# Autodesk Inventor assembly: 40-J4
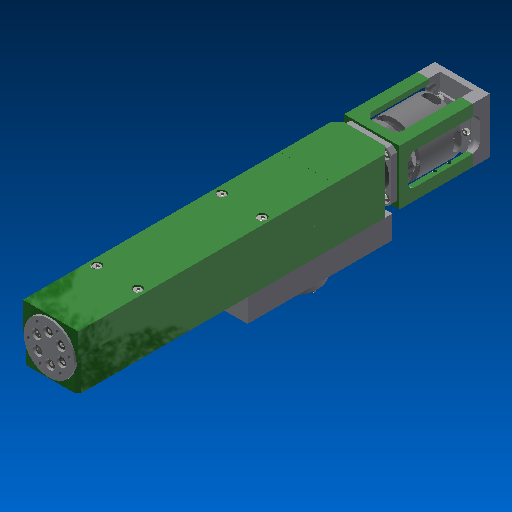
[picture p0: Inventor's stored thumbnail of the model, 512x512]
Saved by Autodesk Inventor 2018 (Build 220112000, 112)
## iProperties
Created: 2020-06-07
Part Number: 40-J4
Document SubType Name: Assembly
Designer: Bunny320
Author: Bunny320
## Documents named in this file (15)
- C:\Users\Bunny320\Desktop\sechs\4-CAD\40-J4.iam
- C:\Users\Bunny320\Desktop\sechs\4-CAD\motor unit 2820.iam
- C:\Users\Bunny320\Desktop\sechs\4-CAD\401-flange.ipt
- C:\Users\Bunny320\Desktop\sechs\4-CAD\402-gearbox-housing.ipt
- C:\Users\Bunny320\Desktop\sechs\4-CAD\403-coupler dummy.ipt
- C:\Users\Bunny320\Desktop\sechs\4-CAD\404-shaft.ipt
- C:\Users\Bunny320\Desktop\sechs\4-CAD\standardParts\Pololu mounting hub\pololu-universal-aluminum-mounting-hub-for-6mm-shaft-m3-holes.ipt
- C:\Users\Bunny320\Desktop\sechs\4-CAD\standardParts\61705-2RZ\W 61705-2RZ.iam
- C:\Users\Bunny320\Desktop\sechs\4-CAD\405-output disk.ipt
- C:\Users\Bunny320\Desktop\sechs\4-CAD\standardParts\W 606-2Z\W 606-2Z.iam
- C:\Users\Bunny320\Desktop\sechs\4-CAD\402-gearbox-housing-cap.ipt
- C:\Users\Bunny320\Documents\Inventor\Content Center Files\R2018\en-US\ISO 10642(2)\ISO 10642  - M3  x  12.ipt
- C:\Users\Bunny320\Documents\Inventor\Content Center Files\R2018\en-US\ISO 4762(1)\DIN EN ISO 4762 - M3 x 25.ipt
- C:\Users\Bunny320\Documents\Inventor\Content Center Files\R2018\en-US\ISO 4762(1)\DIN EN ISO 4762 - M3 x 12.ipt
- C:\Users\Bunny320\Documents\Inventor\Content Center Files\R2018\en-US\ISO 4762(1)\DIN EN ISO 4762 - M3 x 8.ipt
## Components (41 placed, 14 different names)
1. motor unit 2820:1 [sub-assembly] — Flush:1, Flush:2, Flush:3, Mate:1, Mate:2, Mate:3, Mate:5, Mate:12
2. 401-flange:1 — Mate:1, Flush:5, Flush:6, Mate:17, Mate:37, Mate:38, Mate:39, Mate:40, Mate:41, Mate:42, Mate:43, Mate:44, Mate:45, Mate:46, Mate:47, Mate:48, Mate:49, Mate:50, Mate:51, Mate:52, Mate:53, Mate:54, Mate:55, Mate:56, Mate:57, Mate:58, Mate:59, Mate:60, Mate:61, Mate:62, Mate:63, Mate:64, Mate:65, Mate:66, Mate:67, Mate:68
3. 402-gearbox-housing:1 — Mate:2, Mate:3, Flush:5, Flush:6, Mate:20, Mate:22, Flush:8, Mate:23, Mate:24, Mate:25, Mate:26, Mate:27, Mate:28
4. 403-coupler dummy:1 — Mate:5, Mate:6
5. 404-shaft:1 — Mate:6, Mate:7, Flush:7, Mate:12, Mate:19, Mate:21
6. pololu-universal-aluminum-mounting-hub-for-6mm-shaft-m3-holes:1 — Mate:7, Flush:7, Mate:10
7. W 61705-2RZ:1 [sub-assembly] — Mate:10, Mate:11, Mate:18
8. 405-output disk:1 — Mate:11, Mate:17, Mate:18, Mate:69, Mate:70, Mate:71, Mate:72, Mate:73, Mate:74, Mate:75, Mate:76, Mate:77, Mate:78, Mate:79, Mate:80
9. W 606-2Z:1 [sub-assembly] — Mate:19, Mate:20
10. W 606-2Z:2 [sub-assembly] — Mate:21, Mate:22
11. 402-gearbox-housing-cap:1 — Flush:8, Mate:23, Mate:24, Mate:29, Mate:30, Mate:31, Mate:32, Mate:33, Mate:34, Mate:35, Mate:36
12. DIN EN ISO 10642 M3  x  12:1 — Mate:25
13. DIN EN ISO 10642 M3  x  12:2 — Mate:26
14. DIN EN ISO 10642 M3  x  12:3 — Mate:27
15. DIN EN ISO 10642 M3  x  12:4 — Mate:28
16. DIN EN ISO 4762 M3 x 25:1 — Mate:29, Mate:30
17. DIN EN ISO 4762 M3 x 25:2 — Mate:31, Mate:32
18. DIN EN ISO 4762 M3 x 25:3 — Mate:33, Mate:34
19. DIN EN ISO 4762 M3 x 25:4 — Mate:35, Mate:36
20. DIN EN ISO 4762 M3 x 12:1 — Mate:37, Mate:38
21. DIN EN ISO 4762 M3 x 12:2 — Mate:39, Mate:40
22. DIN EN ISO 4762 M3 x 12:3 — Mate:41, Mate:42
23. DIN EN ISO 4762 M3 x 12:4 — Mate:43, Mate:44
24. DIN EN ISO 4762 M3 x 12:5 — Mate:45, Mate:46
25. DIN EN ISO 4762 M3 x 12:6 — Mate:47, Mate:48
26. DIN EN ISO 4762 M3 x 12:7 — Mate:49, Mate:50
27. DIN EN ISO 4762 M3 x 12:8 — Mate:51, Mate:52
28. DIN EN ISO 4762 M3 x 8:1 — Mate:53, Mate:54
29. DIN EN ISO 4762 M3 x 8:2 — Mate:55, Mate:56
30. DIN EN ISO 4762 M3 x 8:3 — Mate:57, Mate:58
31. DIN EN ISO 4762 M3 x 8:4 — Mate:59, Mate:60
32. DIN EN ISO 4762 M3 x 8:5 — Mate:61, Mate:62
33. DIN EN ISO 4762 M3 x 8:6 — Mate:63, Mate:64
34. DIN EN ISO 4762 M3 x 8:7 — Mate:65, Mate:66
35. DIN EN ISO 4762 M3 x 8:8 — Mate:67, Mate:68
36. DIN EN ISO 4762 M3 x 12:9 — Mate:69, Mate:70
37. DIN EN ISO 4762 M3 x 12:10 — Mate:71, Mate:72
38. DIN EN ISO 4762 M3 x 12:11 — Mate:73, Mate:74
39. DIN EN ISO 4762 M3 x 12:12 — Mate:75, Mate:76
40. DIN EN ISO 4762 M3 x 12:13 — Mate:77, Mate:78
41. DIN EN ISO 4762 M3 x 12:14 — Mate:79, Mate:80
## Relationships (80: Mate 73, Flush 7)
- Flush:1: motor unit 2820:1
- Flush:2: motor unit 2820:1
- Flush:3: motor unit 2820:1
- Mate:1: motor unit 2820:1 ↔ 401-flange:1
- Mate:2: motor unit 2820:1 ↔ 402-gearbox-housing:1
- Mate:3: motor unit 2820:1 ↔ 402-gearbox-housing:1
- Flush:5: 401-flange:1 ↔ 402-gearbox-housing:1
- Flush:6: 401-flange:1 ↔ 402-gearbox-housing:1
- Mate:5: motor unit 2820:1 ↔ 403-coupler dummy:1
- Mate:6: 403-coupler dummy:1 ↔ 404-shaft:1
- Mate:7: 404-shaft:1 ↔ pololu-universal-aluminum-mounting-hub-for-6mm-shaft-m3-holes:1
- Flush:7: 404-shaft:1 ↔ pololu-universal-aluminum-mounting-hub-for-6mm-shaft-m3-holes:1
- Mate:10: pololu-universal-aluminum-mounting-hub-for-6mm-shaft-m3-holes:1 ↔ W 61705-2RZ:1
- Mate:11: W 61705-2RZ:1 ↔ 405-output disk:1
- Mate:12 (2 mm): motor unit 2820:1 ↔ 404-shaft:1
- Mate:17 (-168 mm): 401-flange:1 ↔ 405-output disk:1
- Mate:18: W 61705-2RZ:1 ↔ 405-output disk:1
- Mate:19: 404-shaft:1 ↔ W 606-2Z:1
- Mate:20: 402-gearbox-housing:1 ↔ W 606-2Z:1
- Mate:21: 404-shaft:1 ↔ W 606-2Z:2
- Mate:22: 402-gearbox-housing:1 ↔ W 606-2Z:2
- Flush:8: 402-gearbox-housing:1 ↔ 402-gearbox-housing-cap:1
- Mate:23: 402-gearbox-housing:1 ↔ 402-gearbox-housing-cap:1
- Mate:24: 402-gearbox-housing:1 ↔ 402-gearbox-housing-cap:1
- Mate:25: 402-gearbox-housing:1 ↔ DIN EN ISO 10642 M3  x  12:1
- Mate:26: 402-gearbox-housing:1 ↔ DIN EN ISO 10642 M3  x  12:2
- Mate:27: 402-gearbox-housing:1 ↔ DIN EN ISO 10642 M3  x  12:3
- Mate:28: 402-gearbox-housing:1 ↔ DIN EN ISO 10642 M3  x  12:4
- Mate:29: 402-gearbox-housing-cap:1 ↔ DIN EN ISO 4762 M3 x 25:1
- Mate:30: 402-gearbox-housing-cap:1 ↔ DIN EN ISO 4762 M3 x 25:1
- Mate:31: 402-gearbox-housing-cap:1 ↔ DIN EN ISO 4762 M3 x 25:2
- Mate:32: 402-gearbox-housing-cap:1 ↔ DIN EN ISO 4762 M3 x 25:2
- Mate:33: 402-gearbox-housing-cap:1 ↔ DIN EN ISO 4762 M3 x 25:3
- Mate:34: 402-gearbox-housing-cap:1 ↔ DIN EN ISO 4762 M3 x 25:3
- Mate:35: 402-gearbox-housing-cap:1 ↔ DIN EN ISO 4762 M3 x 25:4
- Mate:36: 402-gearbox-housing-cap:1 ↔ DIN EN ISO 4762 M3 x 25:4
- Mate:37: 401-flange:1 ↔ DIN EN ISO 4762 M3 x 12:1
- Mate:38: 401-flange:1 ↔ DIN EN ISO 4762 M3 x 12:1
- Mate:39: 401-flange:1 ↔ DIN EN ISO 4762 M3 x 12:2
- Mate:40: 401-flange:1 ↔ DIN EN ISO 4762 M3 x 12:2
- Mate:41: 401-flange:1 ↔ DIN EN ISO 4762 M3 x 12:3
- Mate:42: 401-flange:1 ↔ DIN EN ISO 4762 M3 x 12:3
- Mate:43: 401-flange:1 ↔ DIN EN ISO 4762 M3 x 12:4
- Mate:44: 401-flange:1 ↔ DIN EN ISO 4762 M3 x 12:4
- Mate:45: 401-flange:1 ↔ DIN EN ISO 4762 M3 x 12:5
- Mate:46: 401-flange:1 ↔ DIN EN ISO 4762 M3 x 12:5
- Mate:47: 401-flange:1 ↔ DIN EN ISO 4762 M3 x 12:6
- Mate:48: 401-flange:1 ↔ DIN EN ISO 4762 M3 x 12:6
- Mate:49: 401-flange:1 ↔ DIN EN ISO 4762 M3 x 12:7
- Mate:50: 401-flange:1 ↔ DIN EN ISO 4762 M3 x 12:7
- Mate:51: 401-flange:1 ↔ DIN EN ISO 4762 M3 x 12:8
- Mate:52: 401-flange:1 ↔ DIN EN ISO 4762 M3 x 12:8
- Mate:53: 401-flange:1 ↔ DIN EN ISO 4762 M3 x 8:1
- Mate:54: 401-flange:1 ↔ DIN EN ISO 4762 M3 x 8:1
- Mate:55: 401-flange:1 ↔ DIN EN ISO 4762 M3 x 8:2
- Mate:56: 401-flange:1 ↔ DIN EN ISO 4762 M3 x 8:2
- Mate:57: 401-flange:1 ↔ DIN EN ISO 4762 M3 x 8:3
- Mate:58: 401-flange:1 ↔ DIN EN ISO 4762 M3 x 8:3
- Mate:59: 401-flange:1 ↔ DIN EN ISO 4762 M3 x 8:4
- Mate:60: 401-flange:1 ↔ DIN EN ISO 4762 M3 x 8:4
- Mate:61: 401-flange:1 ↔ DIN EN ISO 4762 M3 x 8:5
- Mate:62: 401-flange:1 ↔ DIN EN ISO 4762 M3 x 8:5
- Mate:63: 401-flange:1 ↔ DIN EN ISO 4762 M3 x 8:6
- Mate:64: 401-flange:1 ↔ DIN EN ISO 4762 M3 x 8:6
- Mate:65: 401-flange:1 ↔ DIN EN ISO 4762 M3 x 8:7
- Mate:66: 401-flange:1 ↔ DIN EN ISO 4762 M3 x 8:7
- Mate:67: 401-flange:1 ↔ DIN EN ISO 4762 M3 x 8:8
- Mate:68: 401-flange:1 ↔ DIN EN ISO 4762 M3 x 8:8
- Mate:69: 405-output disk:1 ↔ DIN EN ISO 4762 M3 x 12:9
- Mate:70: 405-output disk:1 ↔ DIN EN ISO 4762 M3 x 12:9
- Mate:71: 405-output disk:1 ↔ DIN EN ISO 4762 M3 x 12:10
- Mate:72: 405-output disk:1 ↔ DIN EN ISO 4762 M3 x 12:10
- Mate:73: 405-output disk:1 ↔ DIN EN ISO 4762 M3 x 12:11
- Mate:74: 405-output disk:1 ↔ DIN EN ISO 4762 M3 x 12:11
- Mate:75: 405-output disk:1 ↔ DIN EN ISO 4762 M3 x 12:12
- Mate:76: 405-output disk:1 ↔ DIN EN ISO 4762 M3 x 12:12
- Mate:77: 405-output disk:1 ↔ DIN EN ISO 4762 M3 x 12:13
- Mate:78: 405-output disk:1 ↔ DIN EN ISO 4762 M3 x 12:13
- Mate:79: 405-output disk:1 ↔ DIN EN ISO 4762 M3 x 12:14
- Mate:80: 405-output disk:1 ↔ DIN EN ISO 4762 M3 x 12:14
